# Autodesk Inventor assembly: FE-00004
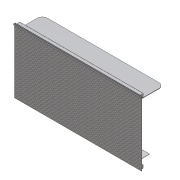
[picture p0: Inventor's stored thumbnail of the model, 180x180]
Saved by Autodesk Inventor 2012 (Build 160160000, 160)
## iProperties
Created: 2008-05-29
Part Number: FE-00004
Document SubType Name: Assembly
Designer: narosenberg
Author: narosenberg
## Documents named in this file (11)
- C:\Data Folder\FRC 2012 Field\Components\FE-00004.iam
- C:\Data Folder\FRC 2012 Field\Components\FE-00004-01.ipt
- C:\Data Folder\FRC 2012 Field\Components\FE-00004-05.ipt
- C:\Data Folder\FRC 2012 Field\Components\FE-00004-04.ipt
- C:\Data Folder\FRC 2012 Field\Components\FE-00004-06.ipt
- C:\Data Folder\FRC 2012 Field\Components\FE-00004-02.iam
- C:\Data Folder\FRC 2012 Field\Components\FE-00004-03.iam
- C:\Data Folder\FRC 2012 Field\Components\FE-00004-08.iam
- C:\Data Folder\FRC 2012 Field\Components\FE-00004-09.ipt
- C:\Data Folder\FRC 2012 Field\Components\FE-00004-07.iam
- C:\Data Folder\FRC 2012 Field\Components\FE-00004-10.ipt
## Components (16 placed, 10 different names)
1. FE-00004-01:1 — Mate:1, Mate:2, Flush:1, Mate:5, Flush:2, Flush:3, Mate:7, Flush:4, Mate:9, Flush:5, Mate:10, Flush:6, Tangent:1, Tangent:2, Mate:20, Mate:21, Mate:22, Flush:8, Flush:9, Mate:23, Flush:10
2. FE-00004-05:1 — Mate:1, Mate:2, Flush:1, Mate:3
3. FE-00004-04:1 — Mate:3, Mate:23, Flush:10
4. FE-00004-06:1 — Mate:5, Flush:2, Flush:3, Mate:6, Mate:8, Mate:11, Mate:12, Mate:14, Mate:16, Mate:17
5. FE-00004-02:1 [sub-assembly] — Mate:6, Mate:7, Flush:4
6. FE-00004-02:2 [sub-assembly] — Mate:8, Mate:9, Flush:5
7. FE-00004-03:1 [sub-assembly] — Mate:10, Mate:11, Flush:6
8. FE-00004-08:1 [sub-assembly] — Mate:13, Mate:14, Flush:7, Mate:21
9. FE-00004-08:2 [sub-assembly] — Mate:17, Mate:18, Mate:19, Mate:20
10. FE-00004-09:1 — Mate:16, Tangent:2, Mate:18, Mate:19
11. FE-00004-09:2 — Mate:12, Tangent:1, Mate:13, Flush:7
12. FE-00004-04:2 — Mate:22, Flush:8, Flush:9, Mate:24, Mate:25, Flush:11, Mate:28, Mate:29, Flush:13
13. FE-00004-07:1 [sub-assembly] — Mate:24, Mate:25, Flush:11, Mate:26, Flush:12, Mate:27
14. FE-00004-07:2 [sub-assembly] — Mate:28, Mate:29, Flush:13, Mate:30, Flush:14, Mate:31
15. FE-00004-10:1 — Mate:26, Flush:12, Mate:27
16. FE-00004-10:2 — Mate:30, Flush:14, Mate:31
## Relationships (45: Mate 29, Flush 14, Tangent 2)
- Mate:1: FE-00004-01:1 ↔ FE-00004-05:1
- Mate:2: FE-00004-01:1 ↔ FE-00004-05:1
- Flush:1: FE-00004-01:1 ↔ FE-00004-05:1
- Mate:3: FE-00004-05:1 ↔ FE-00004-04:1
- Mate:5: FE-00004-01:1 ↔ FE-00004-06:1
- Flush:2 (863.6 mm): FE-00004-01:1 ↔ FE-00004-06:1
- Flush:3 (38.1 mm): FE-00004-01:1 ↔ FE-00004-06:1
- Mate:6: FE-00004-06:1 ↔ FE-00004-02:1
- Mate:7: FE-00004-01:1 ↔ FE-00004-02:1
- Flush:4 (63.5 mm): FE-00004-01:1 ↔ FE-00004-02:1
- Mate:8: FE-00004-06:1 ↔ FE-00004-02:2
- Mate:9: FE-00004-01:1 ↔ FE-00004-02:2
- Flush:5 (63.5 mm): FE-00004-01:1 ↔ FE-00004-02:2
- Mate:10: FE-00004-01:1 ↔ FE-00004-03:1
- Mate:11: FE-00004-06:1 ↔ FE-00004-03:1
- Flush:6 (673.1 mm): FE-00004-01:1 ↔ FE-00004-03:1
- Mate:12: FE-00004-06:1 ↔ FE-00004-09:2
- Tangent:1: FE-00004-01:1 ↔ FE-00004-09:2
- Mate:13: FE-00004-08:1 ↔ FE-00004-09:2
- Mate:14: FE-00004-06:1 ↔ FE-00004-08:1
- Flush:7 (-25.4 mm): FE-00004-08:1 ↔ FE-00004-09:2
- Mate:16: FE-00004-06:1 ↔ FE-00004-09:1
- Tangent:2: FE-00004-01:1 ↔ FE-00004-09:1
- Mate:17: FE-00004-06:1 ↔ FE-00004-08:2
- Mate:18: FE-00004-08:2 ↔ FE-00004-09:1
- Mate:19 (-25.4 mm): FE-00004-08:2 ↔ FE-00004-09:1
- Mate:20 (-557.2125 mm): FE-00004-01:1 ↔ FE-00004-08:2
- Mate:21 (-557.2125 mm): FE-00004-01:1 ↔ FE-00004-08:1
- Mate:22: FE-00004-01:1 ↔ FE-00004-04:2
- Flush:8: FE-00004-01:1 ↔ FE-00004-04:2
- Flush:9 (25.4 mm): FE-00004-01:1 ↔ FE-00004-04:2
- Mate:23: FE-00004-01:1 ↔ FE-00004-04:1
- Flush:10 (25.4 mm): FE-00004-01:1 ↔ FE-00004-04:1
- Mate:24: FE-00004-04:2 ↔ FE-00004-07:1
- Mate:25: FE-00004-04:2 ↔ FE-00004-07:1
- Flush:11 (-127 mm): FE-00004-04:2 ↔ FE-00004-07:1
- Mate:26: FE-00004-07:1 ↔ FE-00004-10:1
- Flush:12: FE-00004-07:1 ↔ FE-00004-10:1
- Mate:27 (-25.4 mm): FE-00004-07:1 ↔ FE-00004-10:1
- Mate:28: FE-00004-04:2 ↔ FE-00004-07:2
- Mate:29: FE-00004-04:2 ↔ FE-00004-07:2
- Flush:13 (127 mm): FE-00004-04:2 ↔ FE-00004-07:2
- Mate:30: FE-00004-07:2 ↔ FE-00004-10:2
- Flush:14: FE-00004-07:2 ↔ FE-00004-10:2
- Mate:31 (-25.4 mm): FE-00004-07:2 ↔ FE-00004-10:2
